# Autodesk Inventor assembly: PPM_Assembly_20251227
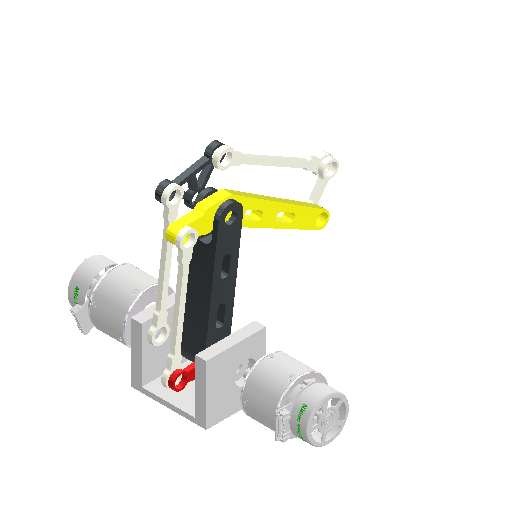
[picture p0: Inventor's stored thumbnail of the model, 512x512]
Saved by Autodesk Inventor 2026.2 (Build 302298000, 298)
## iProperties
Created: 2025-12-27
Part Number: PPM_Assembly_20251227
Document SubType Name: Assembly
Designer: Hsiangyu
Author: Hsiangyu
## Documents named in this file (11)
- C:\Users\Hsiangyu\OneDrive - NTHU\文件\GPA+\20251227\PPM_Assembly_20251227.iam
- C:\Users\Hsiangyu\OneDrive - NTHU\文件\GPA+\20251227\Base.ipt
- C:\Users\Hsiangyu\OneDrive - NTHU\文件\GPA+\Drive\35R52025_20251226.ipt
- C:\Users\Hsiangyu\OneDrive - NTHU\文件\GPA+\20251227\Link_OC.ipt
- C:\Users\Hsiangyu\OneDrive - NTHU\文件\GPA+\20251227\Link_ECH.ipt
- C:\Users\Hsiangyu\OneDrive - NTHU\文件\GPA+\20251227\Link_OD.ipt
- C:\Users\Hsiangyu\OneDrive - NTHU\文件\GPA+\20251227\Link_DE.ipt
- C:\Users\Hsiangyu\OneDrive - NTHU\文件\GPA+\20251227\TriangleLink_CBF.ipt
- C:\Users\Hsiangyu\OneDrive - NTHU\文件\GPA+\20251227\Link_AB.ipt
- C:\Users\Hsiangyu\OneDrive - NTHU\文件\GPA+\20251227\Link_FG.ipt
- C:\Users\Hsiangyu\OneDrive - NTHU\文件\GPA+\20251227\Link_GH.ipt
## Components (11 placed, 10 different names)
1. Base:1 — 齊平:1, 齊平:2, 齊平:3, 貼合:5, 貼合:6, 貼合:13, 貼合:21, 貼合:22, 貼合:23, 貼合:24
2. Link_OC:1 — 貼合:3, 齊平:4, 貼合:5
3. Link_ECH:1 — 貼合:3, 齊平:4, 貼合:8, 貼合:9, 貼合:11, 貼合:17, 貼合:19
4. Link_OD:1 — 貼合:6, 貼合:7, 貼合:10
5. Link_DE:1 — 貼合:7, 貼合:8, 貼合:9, 貼合:10
6. TriangleLink_CBF:1 — 貼合:11, 貼合:12, 貼合:14, 貼合:15, 貼合:20
7. Link_AB:1 — 貼合:12, 貼合:13, 貼合:14
8. Link_FG:1 — 貼合:15, 貼合:16, 貼合:18, 貼合:20
9. Link_GH:1 — 貼合:16, 貼合:17, 貼合:18, 貼合:19
10. 35R52025_20251226:1 — 貼合:21, 貼合:24
11. 35R52025_20251226:2 — 貼合:22, 貼合:23
## Relationships (25: Mate 21, Flush 4)
- 齊平:1 [Flush]: Base:1
- 齊平:2 [Flush]: Base:1
- 齊平:3 [Flush]: Base:1
- 貼合:3 [Mate]: Link_OC:1 ↔ Link_ECH:1
- 齊平:4 [Flush]: Link_OC:1 ↔ Link_ECH:1
- 貼合:5 [Mate]: Base:1 ↔ Link_OC:1
- 貼合:6 [Mate]: Base:1 ↔ Link_OD:1
- 貼合:7 [Mate]: Link_OD:1 ↔ Link_DE:1
- 貼合:8 [Mate]: Link_ECH:1 ↔ Link_DE:1
- 貼合:9 [Mate] (1 mm): Link_ECH:1 ↔ Link_DE:1
- 貼合:10 [Mate] (1 mm): Link_OD:1 ↔ Link_DE:1
- 貼合:11 [Mate]: Link_ECH:1 ↔ TriangleLink_CBF:1
- 貼合:12 [Mate]: TriangleLink_CBF:1 ↔ Link_AB:1
- 貼合:13 [Mate]: Base:1 ↔ Link_AB:1
- 貼合:14 [Mate] (1 mm): TriangleLink_CBF:1 ↔ Link_AB:1
- 貼合:15 [Mate]: TriangleLink_CBF:1 ↔ Link_FG:1
- 貼合:16 [Mate]: Link_FG:1 ↔ Link_GH:1
- 貼合:17 [Mate]: Link_ECH:1 ↔ Link_GH:1
- 貼合:18 [Mate] (1 mm): Link_FG:1 ↔ Link_GH:1
- 貼合:19 [Mate] (1 mm): Link_ECH:1 ↔ Link_GH:1
- 貼合:20 [Mate] (3 mm): TriangleLink_CBF:1 ↔ Link_FG:1
- 貼合:21 [Mate]: Base:1 ↔ 35R52025_20251226:1
- 貼合:22 [Mate]: Base:1 ↔ 35R52025_20251226:2
- 貼合:23 [Mate] (20 mm): Base:1 ↔ 35R52025_20251226:2
- 貼合:24 [Mate] (20 mm): Base:1 ↔ 35R52025_20251226:1
